# Autodesk Inventor assembly: 200-10-ROCKER-BEARING-ASM-01
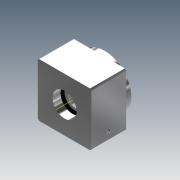
[picture p0: Inventor's stored thumbnail of the model, 180x180]
Saved by Autodesk Inventor 2018.2 (Build 222227000, 227)
## iProperties
Manager: feesmrt
Company: FRANCOR
Created: 2017-10-26
Part Number: 200-10-ROCKER-BEARING-ASM-01
Document SubType Name: Assembly
Designer: feesmrt
Mass: 1761.19 g
Surface Area: 1330.32 cm^2
Volume: 535.142 cm^3
Density: 3.29106 g/cm^3
Project: Rescue Robot
Cost Center: -
Description: Rocker Bearing
Engineer: feesmrt
Authority: feesmrt
Stock Number: 200-10-ROCKER-BEARING-ASM-01
Author: feesmrt
Title: Rocker Bearing
Subject: Rescue Robot
Revision Number: 1
## Documents named in this file (5)
- D:\Programmierung\FRANC0R\CAD\02-Rocker-Bogie-Robot\200-ROCKER-BOGIE\200-10-ROCKER-BEARING\200-10-ROCKER-BEARING-ASM-01.iam
- D:\Programmierung\FRANC0R\CAD\02-Rocker-Bogie-Robot\200-ROCKER-BOGIE\200-10-ROCKER-BEARING\200-10-ROCKER-BEARING-01.ipt
- D:\Programmierung\FRANC0R\CAD\02-Rocker-Bogie-Robot\900-COMPONENTS\900-20-BEARINGS\900-20-BEARINGS-3306-2RS-TN.ipt
- D:\Programmierung\FRANC0R\CAD\02-Rocker-Bogie-Robot\200-ROCKER-BOGIE\200-10-ROCKER-BEARING\200-10-ROCKER-BEARING-02.ipt
- D:\Programmierung\FRANC0R\CAD\02-Rocker-Bogie-Robot\900-COMPONENTS\900-40-SCREWS\900-40-SCREWS-DIN7984_M5x12.ipt
## Components (9 placed, 4 different names)
1. 200-10-ROCKER-BEARING-01:1 — Passend:1, Passend:2, Passend:3, Passend:6, Passend:32
2. 900-20-BEARINGS-3306-2RS-TN:1 — Passend:1, Passend:2, Passend:3, Passend:4
3. 200-10-ROCKER-BEARING-02:1 — Passend:4, Passend:6, Passend:32, Passend:33, Passend:34
4. 900-40-SCREWS-DIN7984_M5x12:1 — Passend:33, Passend:34
5. 900-40-SCREWS-DIN7984_M5x12:2
6. 900-40-SCREWS-DIN7984_M5x12:3
7. 900-40-SCREWS-DIN7984_M5x12:4
8. 900-40-SCREWS-DIN7984_M5x12:5
9. 900-40-SCREWS-DIN7984_M5x12:6
## Component patterns: DIN7984_M5x12 (6 elements)
## Relationships (8: Mate 8)
- Passend:1 [Mate]: 200-10-ROCKER-BEARING-01:1 ↔ 900-20-BEARINGS-3306-2RS-TN:1
- Passend:2 [Mate]: 200-10-ROCKER-BEARING-01:1 ↔ 900-20-BEARINGS-3306-2RS-TN:1
- Passend:3 [Mate]: 200-10-ROCKER-BEARING-01:1 ↔ 900-20-BEARINGS-3306-2RS-TN:1
- Passend:4 [Mate]: 900-20-BEARINGS-3306-2RS-TN:1 ↔ 200-10-ROCKER-BEARING-02:1
- Passend:6 [Mate]: 200-10-ROCKER-BEARING-01:1 ↔ 200-10-ROCKER-BEARING-02:1
- Passend:32 [Mate]: 200-10-ROCKER-BEARING-01:1 ↔ 200-10-ROCKER-BEARING-02:1
- Passend:33 [Mate]: 200-10-ROCKER-BEARING-02:1 ↔ 900-40-SCREWS-DIN7984_M5x12:1
- Passend:34 [Mate]: 200-10-ROCKER-BEARING-02:1 ↔ 900-40-SCREWS-DIN7984_M5x12:1
